# Autodesk Inventor assembly: Sensor_Halterung_Klemme
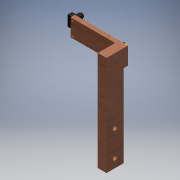
[picture p0: Inventor's stored thumbnail of the model, 180x180]
Saved by Autodesk Inventor 2018 (Build 220112000, 112)
## iProperties
Created: 2018-03-26
Part Number: Sensor_Halterung_Klemme
Material: Generisch
Document SubType Name: Assembly
Designer: Julian
Author: Julian
## Documents named in this file (6)
- C:\Users\Julian\Desktop\Schule\5AHME\Diplomarbeit\Git\fuettr_prototype\Mechanical\Inventorskizzen\Sensor_Halterung_Klemme.iam
- C:\Users\Julian\Desktop\Schule\5AHME\Diplomarbeit\Git\fuettr_prototype\Mechanical\Inventorskizzen\OPB732.ipt
- C:\Users\Julian\Desktop\Schule\5AHME\Diplomarbeit\Git\fuettr_prototype\Mechanical\Inventorskizzen\Sensor_Halterung_Teil1.ipt
- C:\Users\Julian\Desktop\Schule\5AHME\Diplomarbeit\Git\fuettr_prototype\Mechanical\Inventorskizzen\Sensor_Halterung_Teil2ipt.ipt
- C:\Users\Julian\Documents\Inventor\Content Center Files\R2018\de-DE\DIN 96\DIN 96 - 2,5x12.ipt
- C:\Users\Julian\Documents\Inventor\Content Center Files\R2018\de-DE\DIN 96\DIN 96 - 2,5x8.ipt
## Components (7 placed, 5 different names)
1. OPB732:1 — Starr:2, Starr:3, Starr:4
2. Sensor_Halterung_Teil1:1 — Starr:1
3. Sensor_Halterung_Teil2ipt:1 — Starr:1, Starr:2, Starr:5, Starr:6
4. DIN 96 2,5x12:1 — Starr:5
5. DIN 96 2,5x12:2 — Starr:6
6. DIN 96 2,5x8:1 — Starr:3
7. DIN 96 2,5x8:2 — Starr:4
## Relationships (6: WeldJoint 6)
- Starr:1 [WeldJoint]: Sensor_Halterung_Teil1:1 ↔ Sensor_Halterung_Teil2ipt:1
- Starr:2 [WeldJoint]: OPB732:1 ↔ Sensor_Halterung_Teil2ipt:1
- Starr:3 [WeldJoint]: OPB732:1 ↔ DIN 96 2,5x8:1
- Starr:4 [WeldJoint]: OPB732:1 ↔ DIN 96 2,5x8:2
- Starr:5 [WeldJoint]: Sensor_Halterung_Teil2ipt:1 ↔ DIN 96 2,5x12:1
- Starr:6 [WeldJoint]: Sensor_Halterung_Teil2ipt:1 ↔ DIN 96 2,5x12:2
